# Autodesk Inventor assembly: Assembly
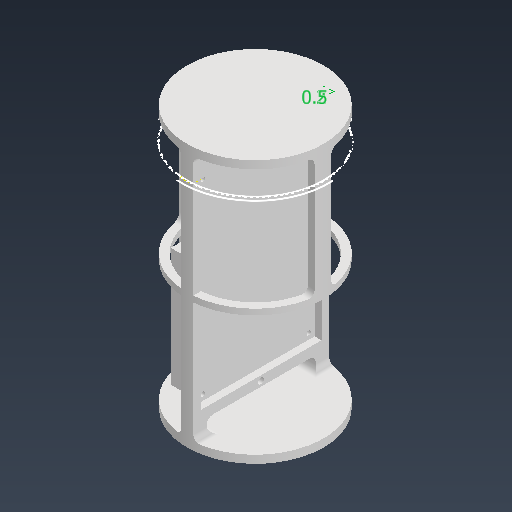
[picture p0: Inventor's stored thumbnail of the model, 512x512]
Saved by Autodesk Inventor 2025.3 (Build 293356000, 356)
## iProperties
Created: 2025-06-10
Part Number: Assembly
Document SubType Name: Assembly
Designer: tolga
Author: tolga
## Documents named in this file (4)
- C:\Users\tolga\Documents\Inventor\Leo_Cansat_v1\Assembly.iam
- C:\Users\tolga\Documents\Inventor\Leo_Cansat_v1\pcb.ipt
- C:\Users\tolga\Documents\Inventor\Leo_Cansat_v1\Frame.ipt
- C:\Users\tolga\Documents\Inventor\Leo_Cansat_v1\battery.ipt
## Components (3 placed, 3 different names)
1. pcb:1 — Flush:1
2. Frame:1 — Flush:1
3. battery:1
## Relationships (1: Flush 1)
- Flush:1: pcb:1 ↔ Frame:1
